# Autodesk Inventor assembly: Assembly1
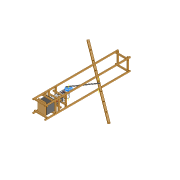
[picture p0: Inventor's stored thumbnail of the model, 180x180]
Saved by Autodesk Inventor 2020 (Build 240168000, 168)
## iProperties
Created: 2022-05-05
Part Number: Assembly1
Document SubType Name: Assembly
Designer: leo
Author: leo
## Documents named in this file (9)
- C:\Users\leo.DESKTOP-592E5E6\Documents\GitHub\TallerDix2022\cad\Inventor\Assembly1.iam
- C:\Users\leo.DESKTOP-592E5E6\Documents\GitHub\TallerDix2022\cad\Inventor\Base listones.ipt
- C:\Users\leo.DESKTOP-592E5E6\Documents\GitHub\TallerDix2022\cad\Inventor\adocreto.ipt
- C:\Users\leo.DESKTOP-592E5E6\Documents\GitHub\TallerDix2022\cad\Inventor\Caja motriz BASE.iam
- C:\Users\leo.DESKTOP-592E5E6\Documents\GitHub\TallerDix2022\cad\Inventor\pieza.ipt
- C:\Users\leo.DESKTOP-592E5E6\Documents\GitHub\TallerDix2022\cad\Inventor\pieza2.ipt
- C:\Users\leo.DESKTOP-592E5E6\Documents\GitHub\TallerDix2022\cad\Inventor\esquema01.ipt
- C:\Users\leo.DESKTOP-592E5E6\Documents\GitHub\TallerDix2022\cad\Inventor\Caja\Poleas dentadas\Poleas de transmision 60Dientes (ZR timing belts).ipt
- C:\Users\leo.DESKTOP-592E5E6\Documents\GitHub\TallerDix2022\cad\Inventor\biela.ipt
## Components (9 placed, 8 different names)
1. esquema01:1 — Flush:4, Flush:5, Flush:6, Mate:7, Mate:8
2. Base listones:1
3. adocreto:1 — Flush:1, Flush:2
4. Caja motriz BASE:1 [sub-assembly] — Flush:3, Flush:7
5. pieza:2 — Mate:2, Insert:1, Insert:3
6. pieza:1 — Mate:5, Mate:6, Insert:2
7. pieza2:1 — Insert:1, Insert:2
8. Poleas de transmision 60Dientes (ZR timing belts):1 — Mate:9, Flush:7, Insert:4
9. biela:1 — Insert:3, Insert:4
## Relationships (20: Flush 7, Mate 7, Insert 4, Angle 2)
- Flush:1: adocreto:1
- Flush:2: adocreto:1
- Flush:3: Caja motriz BASE:1
- Mate:2: pieza:2
- [Mate]: Caja motriz BASE:1 ↔ pieza:2
- Mate:5 (-200 mm): pieza:1
- Mate:6 (1500 mm): pieza:1
- Insert:1 (10 mm): pieza:2 ↔ pieza2:1
- Insert:2 (10 mm): pieza:1 ↔ pieza2:1
- Flush:4: esquema01:1
- Flush:5: esquema01:1
- Flush:6: esquema01:1
- Mate:7: esquema01:1
- Angle:1 (0 deg)
- Mate:8: esquema01:1
- Angle:2 (0 deg)
- Mate:9: Poleas de transmision 60Dientes (ZR timing belts):1
- Flush:7: Caja motriz BASE:1 ↔ Poleas de transmision 60Dientes (ZR timing belts):1
- Insert:3 (5 mm): pieza:2 ↔ biela:1
- Insert:4 (5 mm): Poleas de transmision 60Dientes (ZR timing belts):1 ↔ biela:1
